# Autodesk Inventor assembly: how the new string system would be layed out
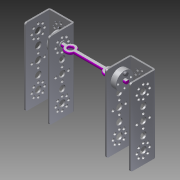
[picture p0: Inventor's stored thumbnail of the model, 180x180]
Saved by Autodesk Inventor 2013 (Build 170138000, 138)
## iProperties
Created: 2014-03-08
Part Number: how the new string system would be layed out
Document SubType Name: Assembly
Designer: kahohbein
Author: kahohbein
## Documents named in this file (5)
- C:\Users\kahohbein\Documents\GitHub\2013-2014_BlockParty\CAD\Lift\MK4\how the new string system would be layed out.iam
- C:\Users\kahohbein\Documents\GitHub\2013-2014_BlockParty\CAD\Lift\MK4\new string management system.ipt
- C:\Users\kahohbein\Documents\GitHub\2013-2014_BlockParty\CAD\COTSParts\Tetrix\Tetrix channel 96mm.ipt
- C:\Users\kahohbein\Documents\GitHub\2013-2014_BlockParty\CAD\COTSParts\Tetrix\Tetrix Hub - axle_MIR.ipt
- C:\Users\kahohbein\Documents\GitHub\2013-2014_BlockParty\CAD\COTSParts\Fasteners\4-40 SHCS x500.ipt
## Components (6 placed, 4 different names)
1. new string management system:2 — Mate:12, Angle:1, Mate:16, Mate:21, Flush:2
2. Tetrix channel 96mm:1 — Mate:4, Flush:1, Mate:5, Mate:20, Mate:22
3. Tetrix channel 96mm:2 — Mate:3, Flush:1, Mate:5, Mate:19, Mate:21
4. Tetrix Hub - axle_MIR:1 — Mate:19, Flush:2
5. Tetrix Hub - axle_MIR:2 — Mate:16, Mate:20, Mate:22, Mate:23, Mate:24
6. 4-40 SHCS x500:1 — Mate:23, Mate:24
## Relationships (14: Mate 11, Flush 2, Angle 1)
- Mate:3: Tetrix channel 96mm:2
- Mate:4: Tetrix channel 96mm:1
- Flush:1: Tetrix channel 96mm:1 ↔ Tetrix channel 96mm:2
- Mate:5 (69.85 mm): Tetrix channel 96mm:1 ↔ Tetrix channel 96mm:2
- Mate:12: new string management system:2
- Angle:1 (90 deg): new string management system:2
- Mate:16: new string management system:2 ↔ Tetrix Hub - axle_MIR:2
- Mate:19: Tetrix channel 96mm:2 ↔ Tetrix Hub - axle_MIR:1
- Mate:20: Tetrix channel 96mm:1 ↔ Tetrix Hub - axle_MIR:2
- Mate:21: new string management system:2 ↔ Tetrix channel 96mm:2
- Mate:22: Tetrix channel 96mm:1 ↔ Tetrix Hub - axle_MIR:2
- Mate:23: Tetrix Hub - axle_MIR:2 ↔ 4-40 SHCS x500:1
- Mate:24: Tetrix Hub - axle_MIR:2 ↔ 4-40 SHCS x500:1
- Flush:2 (-3.175 mm): new string management system:2 ↔ Tetrix Hub - axle_MIR:1
